# Autodesk Inventor assembly: Robot
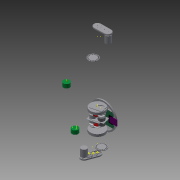
[picture p0: Inventor's stored thumbnail of the model, 180x180]
Saved by Autodesk Inventor 2014 (Build 180170000, 170)
## iProperties
Created: 2013-05-24
Part Number: Robot
Document SubType Name: Assembly
Designer: hartmann
Author: hartmann
## Documents named in this file (9)
- C:\Users\hanse\Desktop\Beep\Hardware\Robot\Robot.iam
- C:\Users\hanse\Desktop\Beep\Hardware\RaspberryPi\RaspberryPi.iam
- C:\Users\hanse\Desktop\Beep\Hardware\Robot\frame.ipt
- C:\Users\hanse\Desktop\Beep\Hardware\Robot\BaneBots2375.ipt
- C:\Users\hanse\Desktop\Beep\Hardware\Model2\motor.ipt
- C:\Users\hanse\Desktop\Beep\Hardware\Z132053\Z.iam
- C:\Users\hanse\Desktop\Beep\Hardware\GetriebeB\Gertiebe.iam
- C:\Users\hanse\Desktop\Beep\Hardware\Robot\EncoderWheel.ipt
- C:\Users\hanse\Desktop\Beep\Hardware\GetriebeB\GetriebeC.iam
## Components (14 placed, 8 different names)
1. RaspberryPi:1 [sub-assembly] — Fluchtend:1
2. frame:1 — Fluchtend:1
3. BaneBots2375:1 — Passend:1, Passend:2, Mate:5, Passend:10, Passend:16
4. BaneBots2375:2 — Passend:1, Passend:3, Mate:6, Passend:11, Passend:15
5. motor:1 — Passend:2, Passend:4, Passend:7, Passend:14
6. motor:2 — Passend:3, Passend:4, Passend:8, Passend:13
7. Z:1 [sub-assembly] — Mate:5
8. Z:2 [sub-assembly] — Mate:6
9. Gertiebe:1 [sub-assembly] — Passend:7, Passend:12, Fluchtend:2
10. Gertiebe:2 [sub-assembly] — Passend:8, Passend:9, Fluchtend:2
11. EncoderWheel:1 — Passend:13
12. EncoderWheel:2 — Passend:14
13. GetriebeC:1 [sub-assembly] — Passend:15
14. GetriebeC:2 [sub-assembly] — Passend:16
## Relationships (18: Mate 16, Flush 2)
- Fluchtend:1 [Flush]: RaspberryPi:1 ↔ frame:1
- Passend:1 [Mate]: BaneBots2375:1 ↔ BaneBots2375:2
- Passend:2 [Mate]: BaneBots2375:1 ↔ motor:1
- Passend:3 [Mate]: BaneBots2375:2 ↔ motor:2
- Passend:4 [Mate]: motor:1 ↔ motor:2
- Mate:5: BaneBots2375:1 ↔ Z:1
- Mate:6: BaneBots2375:2 ↔ Z:2
- Passend:7 [Mate]: motor:1 ↔ Gertiebe:1
- Passend:8 [Mate]: motor:2 ↔ Gertiebe:2
- Passend:9 [Mate]: Gertiebe:2
- Passend:10 [Mate]: BaneBots2375:1
- Passend:11 [Mate]: BaneBots2375:2
- Passend:12 [Mate]: Gertiebe:1
- Fluchtend:2 [Flush]: Gertiebe:1 ↔ Gertiebe:2
- Passend:13 [Mate]: motor:2 ↔ EncoderWheel:1
- Passend:14 [Mate]: motor:1 ↔ EncoderWheel:2
- Passend:15 [Mate]: BaneBots2375:2 ↔ GetriebeC:1
- Passend:16 [Mate]: BaneBots2375:1 ↔ GetriebeC:2
